# Autodesk Inventor assembly: Drone
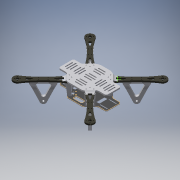
[picture p0: Inventor's stored thumbnail of the model, 180x180]
Saved by Autodesk Inventor 2018 (Build 220112000, 112)
## iProperties
Created: 2019-01-19
Part Number: Drone
Document SubType Name: Assembly
Designer: anirudh
Author: anirudh
## Documents named in this file (6)
- C:\Users\anirudh\Documents\MARS Fund\Drone Stuff\FirstDrone\Drone.iam
- C:\Users\anirudh\Documents\MARS Fund\Drone Stuff\FirstDrone\FlameWheel_F450_Base_Bottom.ipt
- C:\Users\anirudh\Documents\MARS Fund\Drone Stuff\FirstDrone\ArmBracket.ipt
- C:\Users\anirudh\Documents\MARS Fund\Drone Stuff\FirstDrone\MotorLink.ipt
- C:\Users\anirudh\Documents\MARS Fund\Drone Stuff\FirstDrone\TopPlate.ipt
- C:\Users\anirudh\Documents\MARS Fund\Drone Stuff\FirstDrone\LandingGear.ipt
## Components (14 placed, 5 different names)
1. FlameWheel_F450_Base_Bottom:1 — Symmetry:1, Mate:1, Mate:2, Mate:3, Mate:5, Flush:2, Mate:7, Mate:8, Mate:9, Mate:12, Mate:13, Mate:14, Mate:15, Mate:18, Mate:19, Mate:20, Mate:21, Flush:10, Flush:11
2. ArmBracket:1 — Symmetry:1, Mate:1, Mate:2, Mate:3, Flush:1, Mate:4, Mate:6
3. MotorLink:1 — Flush:1, Mate:4, Mate:6, Mate:30, Mate:31, Mate:32
4. ArmBracket:2 — Mate:5, Flush:2, Mate:7, Mate:8, Mate:9, Mate:10, Mate:11, Flush:3
5. MotorLink:2 — Mate:10, Mate:11, Flush:3, Mate:33, Mate:34, Mate:35
6. ArmBracket:3 — Mate:12, Mate:13, Mate:14, Mate:15, Mate:16, Flush:4, Mate:17
7. MotorLink:3 — Mate:16, Flush:4, Mate:17, Mate:29, Mate:36, Mate:37, Mate:38
8. ArmBracket:4 — Mate:18, Mate:19, Mate:20, Mate:21, Mate:22, Flush:5, Mate:23
9. MotorLink:4 — Mate:22, Flush:5, Mate:23, Mate:39, Mate:40, Mate:41
10. TopPlate:1 — Mate:29, Flush:10, Flush:11
11. LandingGear:1 — Mate:36, Mate:37, Mate:38
12. LandingGear:2 — Mate:39, Mate:40, Mate:41
13. LandingGear:3 — Mate:33, Mate:34, Mate:35
14. LandingGear:4 — Mate:30, Mate:31, Mate:32
## Relationships (44: Mate 36, Flush 7, Symmetry 1)
- Symmetry:1: FlameWheel_F450_Base_Bottom:1 ↔ ArmBracket:1
- Mate:1: FlameWheel_F450_Base_Bottom:1 ↔ ArmBracket:1
- Mate:2: FlameWheel_F450_Base_Bottom:1 ↔ ArmBracket:1
- Mate:3: FlameWheel_F450_Base_Bottom:1 ↔ ArmBracket:1
- Flush:1: ArmBracket:1 ↔ MotorLink:1
- Mate:4: ArmBracket:1 ↔ MotorLink:1
- Mate:5: FlameWheel_F450_Base_Bottom:1 ↔ ArmBracket:2
- Mate:6: ArmBracket:1 ↔ MotorLink:1
- Flush:2: FlameWheel_F450_Base_Bottom:1 ↔ ArmBracket:2
- Mate:7: FlameWheel_F450_Base_Bottom:1 ↔ ArmBracket:2
- Mate:8: FlameWheel_F450_Base_Bottom:1 ↔ ArmBracket:2
- Mate:9: FlameWheel_F450_Base_Bottom:1 ↔ ArmBracket:2
- Mate:10: ArmBracket:2 ↔ MotorLink:2
- Mate:11: ArmBracket:2 ↔ MotorLink:2
- Flush:3: ArmBracket:2 ↔ MotorLink:2
- Mate:12: FlameWheel_F450_Base_Bottom:1 ↔ ArmBracket:3
- Mate:13: FlameWheel_F450_Base_Bottom:1 ↔ ArmBracket:3
- Mate:14: FlameWheel_F450_Base_Bottom:1 ↔ ArmBracket:3
- Mate:15: FlameWheel_F450_Base_Bottom:1 ↔ ArmBracket:3
- Mate:16: ArmBracket:3 ↔ MotorLink:3
- Flush:4: ArmBracket:3 ↔ MotorLink:3
- Mate:17: ArmBracket:3 ↔ MotorLink:3
- Mate:18: FlameWheel_F450_Base_Bottom:1 ↔ ArmBracket:4
- Mate:19: FlameWheel_F450_Base_Bottom:1 ↔ ArmBracket:4
- Mate:20: FlameWheel_F450_Base_Bottom:1 ↔ ArmBracket:4
- Mate:21: FlameWheel_F450_Base_Bottom:1 ↔ ArmBracket:4
- Mate:22: ArmBracket:4 ↔ MotorLink:4
- Flush:5: ArmBracket:4 ↔ MotorLink:4
- Mate:23: ArmBracket:4 ↔ MotorLink:4
- Mate:29: MotorLink:3 ↔ TopPlate:1
- Flush:10: FlameWheel_F450_Base_Bottom:1 ↔ TopPlate:1
- Flush:11: FlameWheel_F450_Base_Bottom:1 ↔ TopPlate:1
- Mate:30: MotorLink:1 ↔ LandingGear:4
- Mate:31: MotorLink:1 ↔ LandingGear:4
- Mate:32: MotorLink:1 ↔ LandingGear:4
- Mate:33: MotorLink:2 ↔ LandingGear:3
- Mate:34: MotorLink:2 ↔ LandingGear:3
- Mate:35: MotorLink:2 ↔ LandingGear:3
- Mate:36: MotorLink:3 ↔ LandingGear:1
- Mate:37: MotorLink:3 ↔ LandingGear:1
- Mate:38: MotorLink:3 ↔ LandingGear:1
- Mate:39: MotorLink:4 ↔ LandingGear:2
- Mate:40: MotorLink:4 ↔ LandingGear:2
- Mate:41: MotorLink:4 ↔ LandingGear:2
